# Autodesk Inventor assembly: Bearing
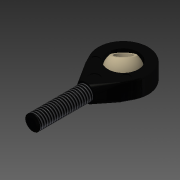
[picture p0: Inventor's stored thumbnail of the model, 180x180]
Saved by Autodesk Inventor 2013 (Build 170138000, 138)
## iProperties
Created: 2014-07-13
Part Number: Bearing
Document SubType Name: Assembly
Designer: User
Author: User
## Documents named in this file (3)
- F:\Exo\Models\3D\External\Bearing.iam
- F:\Exo\Models\3D\External\BearingBall.ipt
- F:\Exo\Models\3D\External\BearingBody.ipt
## Components (2 placed, 2 different names)
1. Ball — Mate:1
2. Body — Mate:1
## Relationships (1: Mate 1)
- Mate:1: Ball ↔ Body
